# Autodesk Inventor assembly: 足回り
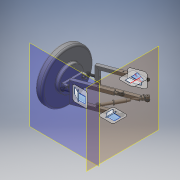
[picture p0: Inventor's stored thumbnail of the model, 180x180]
Saved by Autodesk Inventor 2018 (Build 220112000, 112)
## iProperties
Created: 2017-09-10
Part Number: 足回り
Material: 一般
Document SubType Name: Assembly
Designer: mura5
Author: mura5
## Documents named in this file (9)
- C:\Users\mura5\Documents\RBBR\cart\足回り.iam
- C:\Users\mura5\Documents\RBBR\cart\A.iam
- C:\Users\mura5\Documents\RBBR\cart\車輪取り付け部.iam
- C:\Users\mura5\Documents\RBBR\cart\前輪.ipt
- C:\Users\mura5\Documents\RBBR\cart\前輪シャフト.ipt
- C:\Users\mura5\Documents\RBBR\cart\前輪シャフトワッシャー.ipt
- C:\Users\mura5\Documents\RBBR\cart\M14ワッシャ.ipt
- C:\Users\mura5\Documents\RBBR\cart\hn1_14.ipt
- C:\Users\mura5\Documents\RBBR\cart\スプリング.iam
## Components (11 placed, 8 different names)
1. A:1 [sub-assembly] — 回転:7, 角度:2, フラッシュ:1, 円柱状:1, メイト:1
2. A:2 [sub-assembly] — 回転:6, 角度:2, フラッシュ:1, 回転:15
3. 車輪取り付け部:1 [sub-assembly] — 回転:6, 角度:1, 回転:7, 回転:10, 回転:11, 回転:12
4. 前輪:1 — 回転:8, 回転:9, 正接:1, 角度:3
5. 前輪シャフト:1 — 回転:8
6. 前輪シャフトワッシャー:1 — 回転:9, 回転:10
7. M14ワッシャ:1 — 回転:11, 回転:13
8. M14ワッシャ:2 — 回転:12, 回転:14
9. hn1_14:1 — 回転:13
10. hn1_14:2 — 回転:14
11. スプリング:1 [sub-assembly] — 回転:15, 円柱状:1
## Relationships (17: RevoluteJoint 10, Angle 3, Flush 1, CylindricalJoint 1, Tangent 1, Mate 1)
- 回転:6 [RevoluteJoint]: A:2 ↔ 車輪取り付け部:1
- 角度:1 [Angle] (180 deg): 車輪取り付け部:1
- 回転:7 [RevoluteJoint]: A:1 ↔ 車輪取り付け部:1
- 角度:2 [Angle] (0 deg): A:1 ↔ A:2
- フラッシュ:1 [Flush]: A:1 ↔ A:2
- 回転:8 [RevoluteJoint]: 前輪:1 ↔ 前輪シャフト:1
- 回転:9 [RevoluteJoint]: 前輪:1 ↔ 前輪シャフトワッシャー:1
- 回転:10 [RevoluteJoint]: 車輪取り付け部:1 ↔ 前輪シャフトワッシャー:1
- 回転:11 [RevoluteJoint]: 車輪取り付け部:1 ↔ M14ワッシャ:1
- 回転:12 [RevoluteJoint]: 車輪取り付け部:1 ↔ M14ワッシャ:2
- 回転:13 [RevoluteJoint]: M14ワッシャ:1 ↔ hn1_14:1
- 回転:14 [RevoluteJoint]: M14ワッシャ:2 ↔ hn1_14:2
- 回転:15 [RevoluteJoint]: A:2 ↔ スプリング:1
- 円柱状:1 [CylindricalJoint]: A:1 ↔ スプリング:1
- 正接:1 [Tangent]: 前輪:1
- メイト:1 [Mate]: A:1
- 角度:3 [Angle] (0 deg): 前輪:1
